# Autodesk Inventor assembly: guardrail
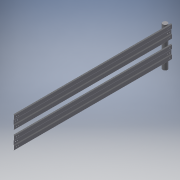
[picture p0: Inventor's stored thumbnail of the model, 180x180]
Saved by Autodesk Inventor 2018 (Build 220112000, 112)
## iProperties
Company: none
Created: 2018-09-19
Part Number: guardrail
Material: 一般
Description: CATIA V5 STEP Exchange
Document SubType Name: Assembly
Designer: ku_sk
Authority: none
Sending System: CATIA V5 STEP AP203
Preprocessor: CATIA Version 5 Release 17 (IN-10)
Title: G:\kuwano\guardrail.stp
Author: none
## Documents named in this file (3)
- D:\Users\ku_sk\Documents\Inventor\ecopaCAD\guardrail.iam
- D:\Users\ku_sk\Documents\Inventor\KS-15 rendering\parts\guardrail_plate.ipt
- D:\Users\ku_sk\Documents\Inventor\KS-15 rendering\parts\guardrail_pole.ipt
## Components (3 placed, 3 different names)
1. guardrail_pole.2 — メイト:1, メイト:2, フラッシュ:1, メイト:3, メイト:4, メイト:5, メイト:6, メイト:7, メイト:8
2. guardrail_plate.1 — メイト:3, メイト:4, メイト:5
3. guardrail_plate.2 — メイト:6, メイト:7, メイト:8
## Relationships (9: Mate 8, Flush 1)
- メイト:1 [Mate]: guardrail_pole.2
- メイト:2 [Mate]: guardrail_pole.2
- フラッシュ:1 [Flush]: guardrail_pole.2
- メイト:3 [Mate]: guardrail_pole.2 ↔ guardrail_plate.1
- メイト:4 [Mate]: guardrail_pole.2 ↔ guardrail_plate.1
- メイト:5 [Mate]: guardrail_pole.2 ↔ guardrail_plate.1
- メイト:6 [Mate]: guardrail_pole.2 ↔ guardrail_plate.2
- メイト:7 [Mate]: guardrail_pole.2 ↔ guardrail_plate.2
- メイト:8 [Mate]: guardrail_pole.2 ↔ guardrail_plate.2
